# Autodesk Inventor assembly: Assembly Arduino Mega RAMPS 1.4
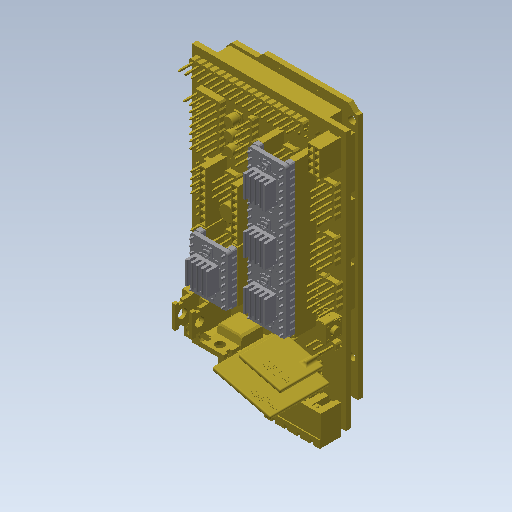
[picture p0: Inventor's stored thumbnail of the model, 512x512]
Saved by Autodesk Inventor 2020 (Build 240168000, 168)
## iProperties
Created: 2018-05-15
Part Number: Assembly Arduino Mega RAMPS 1.4
Document SubType Name: Assembly
Designer: Iulian
Mass: 46.3841 g
Surface Area: 716.146 cm^2
Volume: 46.3841 cm^3
Density: 1 g/cm^3
Description: Arduino-Ramps Assemble
Title: /vol/tmp/translate-3911714334369790748/5afb11f2a5c19511d037ea1c.step
Revision Number: NONE
Subject: 20-1001
## Documents named in this file (3)
- Z:\I.A.B\Proiecte\0008 I.A.B 3D 2.1 Imprimanta aracet Metal\20 Electric\0008-20-01 Assembly Arduino Mega RAMPS 1.4.iam
- Z:\I.A.B\Proiecte\0008 I.A.B 3D 2.1 Imprimanta aracet Metal\20 Electric\User Library-MF-R500___ _________.ipt
- Z:\I.A.B\Proiecte\0008 I.A.B 3D 2.1 Imprimanta aracet Metal\20 Electric\0008-20-1000 Heatsink For A4988.ipt
## Components (5 placed, 2 different names)
1. User Library-MF-R500___ _________.ipt:1 — Mate:1, Mate:2, Mate:3, Mate:4, Mate:6, Flush:3, Flush:4, Mate:7
2. 0005-20-1000 Heatsink For A4988.ipt:2 — Flush:2, Mate:6
3. 0005-20-1000 Heatsink For A4988.ipt:3 — Flush:1, Mate:4, Mate:5, Flush:2
4. 0005-20-1000 Heatsink For A4988.ipt:4 — Mate:1, Mate:2, Mate:3, Flush:1, Mate:5
5. 0005-20-1000 Heatsink For A4988.ipt:5 — Flush:3, Flush:4, Mate:7
## Relationships (11: Mate 7, Flush 4)
- Mate:1: User Library-MF-R500___ _________.ipt:1 ↔ 0005-20-1000 Heatsink For A4988.ipt:4
- Mate:2: User Library-MF-R500___ _________.ipt:1 ↔ 0005-20-1000 Heatsink For A4988.ipt:4
- Mate:3: User Library-MF-R500___ _________.ipt:1 ↔ 0005-20-1000 Heatsink For A4988.ipt:4
- Flush:1: 0005-20-1000 Heatsink For A4988.ipt:3 ↔ 0005-20-1000 Heatsink For A4988.ipt:4
- Mate:4: User Library-MF-R500___ _________.ipt:1 ↔ 0005-20-1000 Heatsink For A4988.ipt:3
- Mate:5: 0005-20-1000 Heatsink For A4988.ipt:3 ↔ 0005-20-1000 Heatsink For A4988.ipt:4
- Flush:2: 0005-20-1000 Heatsink For A4988.ipt:2 ↔ 0005-20-1000 Heatsink For A4988.ipt:3
- Mate:6: User Library-MF-R500___ _________.ipt:1 ↔ 0005-20-1000 Heatsink For A4988.ipt:2
- Flush:3: User Library-MF-R500___ _________.ipt:1 ↔ 0005-20-1000 Heatsink For A4988.ipt:5
- Flush:4: User Library-MF-R500___ _________.ipt:1 ↔ 0005-20-1000 Heatsink For A4988.ipt:5
- Mate:7: User Library-MF-R500___ _________.ipt:1 ↔ 0005-20-1000 Heatsink For A4988.ipt:5
